# Autodesk Inventor assembly: V
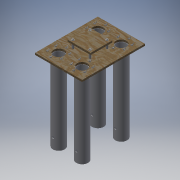
[picture p0: Inventor's stored thumbnail of the model, 180x180]
Saved by Autodesk Inventor 2017 (Build 210142000, 142)
## iProperties
Created: 2016-09-16
Part Number: V
Document SubType Name: Assembly
Designer: Yeash
Author: Yeash
## Documents named in this file (11)
- C:\Users\Yeash\Documents\UCmerced\Q\V.iam
- C:\Users\Yeash\Documents\UCmerced\Q\sheetmappingv5.ipt
- C:\Users\Yeash\Documents\UCmerced\Q\spacer.ipt
- C:\Users\Yeash\Documents\UCmerced\Q\miniplatv3.ipt
- C:\Users\Yeash\Documents\Inventor\Content Center Files\R2017\en-US\ISO 4014(2)\ISO 4014 - M12 x 100 - ISO.ipt
- C:\Users\Yeash\Documents\Inventor\Content Center Files\R2017\en-US\ISO 7089\ISO 7089 - 12 - 140 HV(1).ipt
- C:\Users\Yeash\Documents\Inventor\Content Center Files\R2017\en-US\ISO 4035(2)\ISO 4035 - M12 - ISO.ipt
- C:\Users\Yeash\Documents\UCmerced\Q\flangev6.ipt
- C:\Users\Yeash\Documents\Inventor\Content Center Files\R2017\en-US\ISO 1580\ISO 1580 - M6 x 30.ipt
- C:\Users\Yeash\Documents\Inventor\Content Center Files\R2017\en-US\CNS 4373\CNS 4373 - M 6.ipt
- C:\Users\Yeash\Documents\UCmerced\Q\leg.ipt
## Components (74 placed, 10 different names)
1. sheetmappingv5:1 — Mate:1, Mate:2, Mate:3, Mate:4, Insert:1, Insert:2, Insert:3, Insert:4, Insert:7, Insert:8, Insert:9, Insert:10, Insert:19, Insert:20, Insert:21, Insert:22, Insert:47, Insert:48, Insert:49, Insert:50, Insert:51, Insert:52, Insert:53, Insert:54, Insert:55, Insert:56, Insert:57, Insert:58, Insert:59, Insert:60, Insert:61, Insert:62, Insert:63, Insert:64, Insert:65, Insert:66, Insert:67, Insert:68, Insert:69, Insert:70
2. leg:1 — Insert:72
3. leg:2 — Insert:73
4. leg:3 — Insert:74
5. leg:4 — Mate:5, Insert:71
6. CNS 4373 M 6:23 — Insert:69
7. CNS 4373 M 6:24 — Insert:70
8. CNS 4373 M 6:21 — Insert:67
9. CNS 4373 M 6:20 — Insert:66
10. CNS 4373 M 6:22 — Insert:68
11. CNS 4373 M 6:19 — Insert:65
12. ISO 1580 M6 x 30:24 — Insert:46
13. ISO 1580 M6 x 30:23 — Insert:45
14. ISO 1580 M6 x 30:22 — Insert:44
15. ISO 1580 M6 x 30:21 — Insert:43
16. ISO 1580 M6 x 30:20 — Insert:42
17. ISO 1580 M6 x 30:19 — Insert:41
18. flangev6:1 — Insert:21, Insert:41, Insert:42, Insert:43, Insert:44, Insert:45, Insert:46, Insert:74
19. CNS 4373 M 6:18 — Insert:64
20. CNS 4373 M 6:16 — Insert:62
21. CNS 4373 M 6:17 — Insert:63
22. CNS 4373 M 6:14 — Insert:60
23. CNS 4373 M 6:15 — Insert:61
24. CNS 4373 M 6:13 — Insert:59
25. ISO 1580 M6 x 30:18 — Insert:40
26. ISO 1580 M6 x 30:17 — Insert:39
27. ISO 1580 M6 x 30:16 — Insert:38
28. ISO 1580 M6 x 30:15 — Insert:37
29. ISO 1580 M6 x 30:14 — Insert:36
30. ISO 1580 M6 x 30:13 — Insert:35
31. flangev6:2 — Insert:19, Insert:35, Insert:36, Insert:37, Insert:38, Insert:39, Insert:40, Insert:73
32. CNS 4373 M 6:7 — Insert:53
33. CNS 4373 M 6:6 — Insert:52
34. CNS 4373 M 6:5 — Insert:51
35. CNS 4373 M 6:4 — Insert:50
36. CNS 4373 M 6:2 — Insert:48
37. CNS 4373 M 6:3 — Insert:49
38. ISO 1580 M6 x 30:12 — Insert:34
39. ISO 1580 M6 x 30:11 — Insert:33
40. ISO 1580 M6 x 30:10 — Insert:32
41. ISO 1580 M6 x 30:9 — Insert:31
42. ISO 1580 M6 x 30:8 — Insert:30
43. ISO 1580 M6 x 30:7 — Insert:29
44. flangev6:3 — Insert:20, Insert:29, Insert:30, Insert:31, Insert:32, Insert:33, Insert:34, Mate:5, Insert:71
45. CNS 4373 M 6:12 — Insert:58
46. CNS 4373 M 6:11 — Insert:57
47. CNS 4373 M 6:10 — Insert:56
48. CNS 4373 M 6:9 — Insert:55
49. CNS 4373 M 6:8 — Insert:54
50. CNS 4373 M 6:1 — Insert:47
51. ISO 1580 M6 x 30:4 — Insert:26
52. ISO 1580 M6 x 30:5 — Insert:27
53. ISO 1580 M6 x 30:6 — Insert:28
54. ISO 1580 M6 x 30:3 — Insert:25
55. ISO 1580 M6 x 30:2 — Insert:24
56. ISO 1580 M6 x 30:1 — Insert:23
57. flangev6:4 — Insert:22, Insert:23, Insert:24, Insert:25, Insert:26, Insert:27, Insert:28, Insert:72
58. spacer:1 — Mate:1, Insert:1, Insert:6
59. spacer:2 — Mate:4, Insert:2
60. spacer:3 — Mate:3, Insert:3
61. spacer:4 — Mate:2, Insert:4, Insert:5
62. miniplatv3:1 — Insert:5, Insert:6, Insert:11, Insert:12, Insert:13, Insert:14
63. ISO 4014 M12 x 100:1 — Insert:7
64. ISO 4014 M12 x 100:2 — Insert:8
65. ISO 4014 M12 x 100:3 — Insert:9
66. ISO 4014 M12 x 100:4 — Insert:10
67. ISO 7089 12:1 — Insert:11, Insert:16
68. ISO 7089 12:2 — Insert:12, Insert:17
69. ISO 7089 12:3 — Insert:13, Insert:15
70. ISO 7089 12:4 — Insert:14, Insert:18
71. ISO 4035 M12:1 — Insert:15
72. ISO 4035 M12:2 — Insert:16
73. ISO 4035 M12:3 — Insert:17
74. ISO 4035 M12:4 — Insert:18
## Relationships (79: Insert 74, Mate 5)
- Mate:1: sheetmappingv5:1 ↔ spacer:1
- Mate:2: sheetmappingv5:1 ↔ spacer:4
- Mate:3: sheetmappingv5:1 ↔ spacer:3
- Mate:4: sheetmappingv5:1 ↔ spacer:2
- Insert:1: sheetmappingv5:1 ↔ spacer:1
- Insert:2: sheetmappingv5:1 ↔ spacer:2
- Insert:3: sheetmappingv5:1 ↔ spacer:3
- Insert:4: sheetmappingv5:1 ↔ spacer:4
- Insert:5: spacer:4 ↔ miniplatv3:1
- Insert:6: spacer:1 ↔ miniplatv3:1
- Insert:7: sheetmappingv5:1 ↔ ISO 4014 M12 x 100:1
- Insert:8: sheetmappingv5:1 ↔ ISO 4014 M12 x 100:2
- Insert:9: sheetmappingv5:1 ↔ ISO 4014 M12 x 100:3
- Insert:10: sheetmappingv5:1 ↔ ISO 4014 M12 x 100:4
- Insert:11: miniplatv3:1 ↔ ISO 7089 12:1
- Insert:12: miniplatv3:1 ↔ ISO 7089 12:2
- Insert:13: miniplatv3:1 ↔ ISO 7089 12:3
- Insert:14: miniplatv3:1 ↔ ISO 7089 12:4
- Insert:15: ISO 7089 12:3 ↔ ISO 4035 M12:1
- Insert:16: ISO 7089 12:1 ↔ ISO 4035 M12:2
- Insert:17: ISO 7089 12:2 ↔ ISO 4035 M12:3
- Insert:18: ISO 7089 12:4 ↔ ISO 4035 M12:4
- Insert:19: sheetmappingv5:1 ↔ flangev6:2
- Insert:20: sheetmappingv5:1 ↔ flangev6:3
- Insert:21: sheetmappingv5:1 ↔ flangev6:1
- Insert:22: sheetmappingv5:1 ↔ flangev6:4
- Insert:23: ISO 1580 M6 x 30:1 ↔ flangev6:4
- Insert:24: ISO 1580 M6 x 30:2 ↔ flangev6:4
- Insert:25: ISO 1580 M6 x 30:3 ↔ flangev6:4
- Insert:26: ISO 1580 M6 x 30:4 ↔ flangev6:4
- Insert:27: ISO 1580 M6 x 30:5 ↔ flangev6:4
- Insert:28: ISO 1580 M6 x 30:6 ↔ flangev6:4
- Insert:29: ISO 1580 M6 x 30:7 ↔ flangev6:3
- Insert:30: ISO 1580 M6 x 30:8 ↔ flangev6:3
- Insert:31: ISO 1580 M6 x 30:9 ↔ flangev6:3
- Insert:32: ISO 1580 M6 x 30:10 ↔ flangev6:3
- Insert:33: ISO 1580 M6 x 30:11 ↔ flangev6:3
- Insert:34: ISO 1580 M6 x 30:12 ↔ flangev6:3
- Insert:35: ISO 1580 M6 x 30:13 ↔ flangev6:2
- Insert:36: ISO 1580 M6 x 30:14 ↔ flangev6:2
- Insert:37: ISO 1580 M6 x 30:15 ↔ flangev6:2
- Insert:38: ISO 1580 M6 x 30:16 ↔ flangev6:2
- Insert:39: ISO 1580 M6 x 30:17 ↔ flangev6:2
- Insert:40: ISO 1580 M6 x 30:18 ↔ flangev6:2
- Insert:41: ISO 1580 M6 x 30:19 ↔ flangev6:1
- Insert:42: ISO 1580 M6 x 30:20 ↔ flangev6:1
- Insert:43: ISO 1580 M6 x 30:21 ↔ flangev6:1
- Insert:44: ISO 1580 M6 x 30:22 ↔ flangev6:1
- Insert:45: ISO 1580 M6 x 30:23 ↔ flangev6:1
- Insert:46: ISO 1580 M6 x 30:24 ↔ flangev6:1
- Insert:47: sheetmappingv5:1 ↔ CNS 4373 M 6:1
- Insert:48: sheetmappingv5:1 ↔ CNS 4373 M 6:2
- Insert:49: sheetmappingv5:1 ↔ CNS 4373 M 6:3
- Insert:50: sheetmappingv5:1 ↔ CNS 4373 M 6:4
- Insert:51: sheetmappingv5:1 ↔ CNS 4373 M 6:5
- Insert:52: sheetmappingv5:1 ↔ CNS 4373 M 6:6
- Insert:53: sheetmappingv5:1 ↔ CNS 4373 M 6:7
- Insert:54: sheetmappingv5:1 ↔ CNS 4373 M 6:8
- Insert:55: sheetmappingv5:1 ↔ CNS 4373 M 6:9
- Insert:56: sheetmappingv5:1 ↔ CNS 4373 M 6:10
- Insert:57: sheetmappingv5:1 ↔ CNS 4373 M 6:11
- Insert:58: sheetmappingv5:1 ↔ CNS 4373 M 6:12
- Insert:59: sheetmappingv5:1 ↔ CNS 4373 M 6:13
- Insert:60: sheetmappingv5:1 ↔ CNS 4373 M 6:14
- Insert:61: sheetmappingv5:1 ↔ CNS 4373 M 6:15
- Insert:62: sheetmappingv5:1 ↔ CNS 4373 M 6:16
- Insert:63: sheetmappingv5:1 ↔ CNS 4373 M 6:17
- Insert:64: sheetmappingv5:1 ↔ CNS 4373 M 6:18
- Insert:65: sheetmappingv5:1 ↔ CNS 4373 M 6:19
- Insert:66: sheetmappingv5:1 ↔ CNS 4373 M 6:20
- Insert:67: sheetmappingv5:1 ↔ CNS 4373 M 6:21
- Insert:68: sheetmappingv5:1 ↔ CNS 4373 M 6:22
- Insert:69: sheetmappingv5:1 ↔ CNS 4373 M 6:23
- Insert:70: sheetmappingv5:1 ↔ CNS 4373 M 6:24
- Mate:5: leg:4 ↔ flangev6:3
- Insert:71: leg:4 ↔ flangev6:3
- Insert:72: leg:1 ↔ flangev6:4
- Insert:73: leg:2 ↔ flangev6:2
- Insert:74: leg:3 ↔ flangev6:1
